# Autodesk Inventor assembly: Shooter Curve Assembly
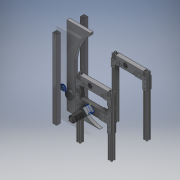
[picture p0: Inventor's stored thumbnail of the model, 180x180]
Saved by Autodesk Inventor 2018 (Build 220112000, 112)
## iProperties
Created: 2020-02-01
Part Number: Shooter Curve Assembly
Document SubType Name: Assembly
Designer: Weeb No1
Author: Weeb No1
## Documents named in this file (12)
- C:\Users\T3500STATIC\Documents\GitHub\2020CAD\Gabriel Inventor Files (Shooter, Drivebase)\Shooter Curve Assembly\Main Assembly File\Shooter Curve Assembly.iam
- C:\Users\T3500STATIC\Documents\GitHub\2020CAD\Gabriel Inventor Files (Shooter, Drivebase)\Shooter Curve Assembly\Part Files\Shooter Main Curve.ipt
- C:\Users\T3500STATIC\Documents\GitHub\2020CAD\Gabriel Inventor Files (Shooter, Drivebase)\Shooter Curve Assembly\Part Files\8020 1010 x 15.ipt
- C:\Users\T3500STATIC\Documents\GitHub\2020CAD\Gabriel Inventor Files (Shooter, Drivebase)\Shooter Curve Assembly\Part Files\1x2 5 in Beam Flywheel Mount.ipt
- C:\Users\T3500STATIC\Documents\GitHub\2020CAD\Over bumper intake\Parts\VersaPlanetary_v2_Single_Stage_10_1_with_775_Series.iam
- C:\Users\T3500STATIC\Documents\GitHub\2020CAD\Gabriel Inventor Files (Shooter, Drivebase)\Shooter Curve Assembly\Part Files\1x2 7 in Beam Motor Mount.ipt
- C:\Users\T3500STATIC\Documents\GitHub\2020CAD\Gabriel Inventor Files (Shooter, Drivebase)\Gussets\L-Gusset 3 Hole 0.25in Hole.ipt
- C:\Users\T3500STATIC\Documents\GitHub\2020CAD\Gabriel Inventor Files (Shooter, Drivebase)\Shooter Curve Assembly\Part Files\1x1 20 in Curve Support Beam.ipt
- C:\Users\T3500STATIC\Documents\GitHub\2020CAD\Gabriel Inventor Files (Shooter, Drivebase)\Gussets\L-Guesset 4 Hole 0.25in Hole.ipt
- C:\Users\T3500STATIC\Documents\GitHub\2020CAD\Gabriel Inventor Files (Shooter, Drivebase)\Gussets\L-Guesset 5 Hole 0.25in Hole.ipt
- C:\Users\T3500STATIC\Documents\GitHub\2020CAD\Gabriel Inventor Files (Shooter, Drivebase)\Shooter Curve Assembly\Part Files\_18t_Aluminum_Hub_Sprocket_25_Chain_1_2_Hex_Bore_217-3488.ipt
- C:\Users\T3500STATIC\Documents\GitHub\2020CAD\Gabriel Inventor Files (Shooter, Drivebase)\Shooter Curve Assembly\Part Files\2_OD_Straight_Flex_Wheel_217-6354.ipt
## Components (32 placed, 11 different names)
1. Shooter Main Curve:1 — Flush:1, Mate:1, Mate:2, Flush:2, Flush:3, Flush:18, Flush:20, Mate:68, Flush:36, Flush:37, Flush:40, Flush:41, Mate:133
2. 8020 1010 x 15:1 — Flush:1, Mate:1, Flush:5, Flush:6, Mate:7, Flush:11, Flush:14, Flush:18, Flush:23, Flush:24, Mate:51, Mate:56, Mate:60, Mate:82, Mate:85, Mate:97, Mate:100
3. 8020 1010 x 15:2 — Flush:4, Mate:3, Flush:7, Mate:9, Flush:15, Flush:19, Flush:22, Flush:25, Mate:127, Mate:130
4. Shooter Main Curve:2 — Mate:2, Flush:2, Flush:3, Flush:4, Mate:3, Flush:19, Flush:21, Mate:67, Flush:35, Flush:38, Flush:39, Mate:132
5. 8020 1010 x 15:3 — Flush:5, Flush:6, Flush:10, Flush:12, Flush:13, Flush:20, Mate:11, Flush:23, Mate:50, Flush:34, Mate:63, Mate:65, Mate:89, Mate:93, Mate:103, Mate:123
6. 8020 1010 x 15:4 — Flush:7, Flush:10, Flush:17, Flush:21, Mate:10, Flush:22, Mate:107, Mate:111
7. 1x2 5 in Beam Flywheel Mount:1 — Mate:9, Flush:15, Flush:17, Mate:10, Flush:25, Mate:106, Mate:108, Mate:109, Mate:110, Mate:112, Mate:113, Mate:126, Mate:128, Mate:129, Mate:131
8. 1x2 5 in Beam Flywheel Mount:2 — Mate:7, Flush:11, Flush:12, Flush:13, Flush:14, Mate:11, Flush:24, Mate:55, Mate:57, Mate:58, Mate:59, Mate:61, Mate:62, Mate:64, Mate:66
9. VersaPlanetary_v2_Single_Stage_10_1_with_775_Series:1 [sub-assembly] — Mate:52, Mate:53, Mate:54
10. 1x2 7 in Beam Motor Mount:1 — Mate:50, Mate:51, Flush:34, Mate:52, Mate:53, Mate:54, Mate:81, Mate:83, Mate:86, Mate:87, Mate:88, Mate:90, Mate:91, Mate:92, Mate:94, Mate:95, Mate:96, Mate:98, Mate:99, Mate:101, Mate:102, Mate:104, Mate:105, Mate:122, Mate:124, Mate:125
11. L-Gusset 3 Hole 0.25in Hole:1 — Mate:61, Mate:62, Mate:63
12. L-Gusset 3 Hole 0.25in Hole:2 — Mate:55, Mate:56, Mate:57
13. L-Gusset 3 Hole 0.25in Hole:3 — Mate:58, Mate:59, Mate:60
14. L-Gusset 3 Hole 0.25in Hole:4 — Mate:64, Mate:65, Mate:66
15. 1x1 20 in Curve Support Beam:1 — Mate:68, Flush:36, Flush:37
16. 1x1 20 in Curve Support Beam:2 — Mate:67, Flush:35, Flush:38
17. L-Guesset 4 Hole 0.25in Hole:3 — Mate:88, Mate:89, Mate:90, Mate:91
18. L-Guesset 4 Hole 0.25in Hole:5 — Mate:81, Mate:82, Mate:83
19. L-Guesset 4 Hole 0.25in Hole:6 — Mate:85, Mate:86, Mate:87
20. L-Guesset 4 Hole 0.25in Hole:9 — Mate:92, Mate:93, Mate:94, Mate:95
21. L-Gusset 3 Hole 0.25in Hole:9 — Mate:96, Mate:97, Mate:98
22. L-Gusset 3 Hole 0.25in Hole:10 — Mate:99, Mate:100, Mate:101
23. L-Guesset 5 Hole 0.25in Hole:1 — Mate:102, Mate:103, Mate:104, Mate:105
24. L-Guesset 5 Hole 0.25in Hole:2 — Mate:110, Mate:111, Mate:112, Mate:113
25. L-Guesset 5 Hole 0.25in Hole:3 — Mate:106, Mate:107, Mate:108, Mate:109
26. L-Guesset 5 Hole 0.25in Hole:6 — Mate:122, Mate:123, Mate:124, Mate:125
27. L-Gusset 3 Hole 0.25in Hole:11 — Mate:126, Mate:127, Mate:128
28. L-Gusset 3 Hole 0.25in Hole:12 — Mate:129, Mate:130, Mate:131
29. _18t_Aluminum_Hub_Sprocket_25_Chain_1_2_Hex_Bore_217-3488:1
30. Shooter Main Curve:4 — Flush:39, Flush:40, Flush:41, Mate:132, Mate:133
31. 2_OD_Straight_Flex_Wheel_217-6354:1
32. 2_OD_Straight_Flex_Wheel_217-6354:2
## Relationships (100: Mate 70, Flush 30)
- Flush:1 (177.8 mm): Shooter Main Curve:1 ↔ 8020 1010 x 15:1
- Mate:1 (25.4 mm): Shooter Main Curve:1 ↔ 8020 1010 x 15:1
- Mate:2 (114.3 mm): Shooter Main Curve:1 ↔ Shooter Main Curve:2
- Flush:2: Shooter Main Curve:1 ↔ Shooter Main Curve:2
- Flush:3: Shooter Main Curve:1 ↔ Shooter Main Curve:2
- Flush:4 (177.8 mm): 8020 1010 x 15:2 ↔ Shooter Main Curve:2
- Mate:3 (25.4 mm): 8020 1010 x 15:2 ↔ Shooter Main Curve:2
- Flush:5: 8020 1010 x 15:1 ↔ 8020 1010 x 15:3
- Flush:6: 8020 1010 x 15:1 ↔ 8020 1010 x 15:3
- Flush:7: 8020 1010 x 15:2 ↔ 8020 1010 x 15:4
- Flush:10: 8020 1010 x 15:3 ↔ 8020 1010 x 15:4
- Mate:7: 8020 1010 x 15:1 ↔ 1x2 5 in Beam Flywheel Mount:2
- Flush:11: 8020 1010 x 15:1 ↔ 1x2 5 in Beam Flywheel Mount:2
- Flush:12: 8020 1010 x 15:3 ↔ 1x2 5 in Beam Flywheel Mount:2
- Flush:13: 8020 1010 x 15:3 ↔ 1x2 5 in Beam Flywheel Mount:2
- Flush:14: 8020 1010 x 15:1 ↔ 1x2 5 in Beam Flywheel Mount:2
- Mate:9: 8020 1010 x 15:2 ↔ 1x2 5 in Beam Flywheel Mount:1
- Flush:15: 8020 1010 x 15:2 ↔ 1x2 5 in Beam Flywheel Mount:1
- Flush:17: 8020 1010 x 15:4 ↔ 1x2 5 in Beam Flywheel Mount:1
- Flush:18 (-25.4 mm): Shooter Main Curve:1 ↔ 8020 1010 x 15:1
- Flush:19 (-25.4 mm): 8020 1010 x 15:2 ↔ Shooter Main Curve:2
- Flush:20 (-25.4 mm): Shooter Main Curve:1 ↔ 8020 1010 x 15:3
- Flush:21 (-25.4 mm): Shooter Main Curve:2 ↔ 8020 1010 x 15:4
- Mate:10: 8020 1010 x 15:4 ↔ 1x2 5 in Beam Flywheel Mount:1
- Mate:11: 8020 1010 x 15:3 ↔ 1x2 5 in Beam Flywheel Mount:2
- Flush:22: 8020 1010 x 15:2 ↔ 8020 1010 x 15:4
- Flush:23: 8020 1010 x 15:1 ↔ 8020 1010 x 15:3
- Flush:24: 8020 1010 x 15:1 ↔ 1x2 5 in Beam Flywheel Mount:2
- Flush:25: 8020 1010 x 15:2 ↔ 1x2 5 in Beam Flywheel Mount:1
- Mate:50: 8020 1010 x 15:3 ↔ 1x2 7 in Beam Motor Mount:1
- Mate:51: 8020 1010 x 15:1 ↔ 1x2 7 in Beam Motor Mount:1
- Flush:34: 8020 1010 x 15:3 ↔ 1x2 7 in Beam Motor Mount:1
- Mate:52: VersaPlanetary_v2_Single_Stage_10_1_with_775_Series:1 ↔ 1x2 7 in Beam Motor Mount:1
- Mate:53: VersaPlanetary_v2_Single_Stage_10_1_with_775_Series:1 ↔ 1x2 7 in Beam Motor Mount:1
- Mate:54: VersaPlanetary_v2_Single_Stage_10_1_with_775_Series:1 ↔ 1x2 7 in Beam Motor Mount:1
- Mate:55: 1x2 5 in Beam Flywheel Mount:2 ↔ L-Gusset 3 Hole 0.25in Hole:2
- Mate:56: 8020 1010 x 15:1 ↔ L-Gusset 3 Hole 0.25in Hole:2
- Mate:57: 1x2 5 in Beam Flywheel Mount:2 ↔ L-Gusset 3 Hole 0.25in Hole:2
- Mate:58: 1x2 5 in Beam Flywheel Mount:2 ↔ L-Gusset 3 Hole 0.25in Hole:3
- Mate:59: 1x2 5 in Beam Flywheel Mount:2 ↔ L-Gusset 3 Hole 0.25in Hole:3
- Mate:60: 8020 1010 x 15:1 ↔ L-Gusset 3 Hole 0.25in Hole:3
- Mate:61: 1x2 5 in Beam Flywheel Mount:2 ↔ L-Gusset 3 Hole 0.25in Hole:1
- Mate:62: 1x2 5 in Beam Flywheel Mount:2 ↔ L-Gusset 3 Hole 0.25in Hole:1
- Mate:63: 8020 1010 x 15:3 ↔ L-Gusset 3 Hole 0.25in Hole:1
- Mate:64: 1x2 5 in Beam Flywheel Mount:2 ↔ L-Gusset 3 Hole 0.25in Hole:4
- Mate:65: 8020 1010 x 15:3 ↔ L-Gusset 3 Hole 0.25in Hole:4
- Mate:66: 1x2 5 in Beam Flywheel Mount:2 ↔ L-Gusset 3 Hole 0.25in Hole:4
- Mate:67: Shooter Main Curve:2 ↔ 1x1 20 in Curve Support Beam:2
- Flush:35 (-25.4 mm): Shooter Main Curve:2 ↔ 1x1 20 in Curve Support Beam:2
- Mate:68: Shooter Main Curve:1 ↔ 1x1 20 in Curve Support Beam:1
- Flush:36 (-25.4 mm): Shooter Main Curve:1 ↔ 1x1 20 in Curve Support Beam:1
- Flush:37: Shooter Main Curve:1 ↔ 1x1 20 in Curve Support Beam:1
- Flush:38: Shooter Main Curve:2 ↔ 1x1 20 in Curve Support Beam:2
- Mate:81: 1x2 7 in Beam Motor Mount:1 ↔ L-Guesset 4 Hole 0.25in Hole:5
- Mate:82: 8020 1010 x 15:1 ↔ L-Guesset 4 Hole 0.25in Hole:5
- Mate:83: 1x2 7 in Beam Motor Mount:1 ↔ L-Guesset 4 Hole 0.25in Hole:5
- Mate:85: 8020 1010 x 15:1 ↔ L-Guesset 4 Hole 0.25in Hole:6
- Mate:86: 1x2 7 in Beam Motor Mount:1 ↔ L-Guesset 4 Hole 0.25in Hole:6
- Mate:87: 1x2 7 in Beam Motor Mount:1 ↔ L-Guesset 4 Hole 0.25in Hole:6
- Mate:88: 1x2 7 in Beam Motor Mount:1 ↔ L-Guesset 4 Hole 0.25in Hole:3
- Mate:89: 8020 1010 x 15:3 ↔ L-Guesset 4 Hole 0.25in Hole:3
- Mate:90: 1x2 7 in Beam Motor Mount:1 ↔ L-Guesset 4 Hole 0.25in Hole:3
- Mate:91: 1x2 7 in Beam Motor Mount:1 ↔ L-Guesset 4 Hole 0.25in Hole:3
- Mate:92: 1x2 7 in Beam Motor Mount:1 ↔ L-Guesset 4 Hole 0.25in Hole:9
- Mate:93: 8020 1010 x 15:3 ↔ L-Guesset 4 Hole 0.25in Hole:9
- Mate:94: 1x2 7 in Beam Motor Mount:1 ↔ L-Guesset 4 Hole 0.25in Hole:9
- Mate:95: 1x2 7 in Beam Motor Mount:1 ↔ L-Guesset 4 Hole 0.25in Hole:9
- Mate:96: 1x2 7 in Beam Motor Mount:1 ↔ L-Gusset 3 Hole 0.25in Hole:9
- Mate:97: 8020 1010 x 15:1 ↔ L-Gusset 3 Hole 0.25in Hole:9
- Mate:98: 1x2 7 in Beam Motor Mount:1 ↔ L-Gusset 3 Hole 0.25in Hole:9
- Mate:99: 1x2 7 in Beam Motor Mount:1 ↔ L-Gusset 3 Hole 0.25in Hole:10
- Mate:100: 8020 1010 x 15:1 ↔ L-Gusset 3 Hole 0.25in Hole:10
- Mate:101: 1x2 7 in Beam Motor Mount:1 ↔ L-Gusset 3 Hole 0.25in Hole:10
- Mate:102: 1x2 7 in Beam Motor Mount:1 ↔ L-Guesset 5 Hole 0.25in Hole:1
- Mate:103: 8020 1010 x 15:3 ↔ L-Guesset 5 Hole 0.25in Hole:1
- Mate:104: 1x2 7 in Beam Motor Mount:1 ↔ L-Guesset 5 Hole 0.25in Hole:1
- Mate:105: 1x2 7 in Beam Motor Mount:1 ↔ L-Guesset 5 Hole 0.25in Hole:1
- Mate:106: 1x2 5 in Beam Flywheel Mount:1 ↔ L-Guesset 5 Hole 0.25in Hole:3
- Mate:107: 8020 1010 x 15:4 ↔ L-Guesset 5 Hole 0.25in Hole:3
- Mate:108: 1x2 5 in Beam Flywheel Mount:1 ↔ L-Guesset 5 Hole 0.25in Hole:3
- Mate:109: 1x2 5 in Beam Flywheel Mount:1 ↔ L-Guesset 5 Hole 0.25in Hole:3
- Mate:110: 1x2 5 in Beam Flywheel Mount:1 ↔ L-Guesset 5 Hole 0.25in Hole:2
- Mate:111: 8020 1010 x 15:4 ↔ L-Guesset 5 Hole 0.25in Hole:2
- Mate:112: 1x2 5 in Beam Flywheel Mount:1 ↔ L-Guesset 5 Hole 0.25in Hole:2
- Mate:113: 1x2 5 in Beam Flywheel Mount:1 ↔ L-Guesset 5 Hole 0.25in Hole:2
- Mate:122: 1x2 7 in Beam Motor Mount:1 ↔ L-Guesset 5 Hole 0.25in Hole:6
- Mate:123: 8020 1010 x 15:3 ↔ L-Guesset 5 Hole 0.25in Hole:6
- Mate:124: 1x2 7 in Beam Motor Mount:1 ↔ L-Guesset 5 Hole 0.25in Hole:6
- Mate:125: 1x2 7 in Beam Motor Mount:1 ↔ L-Guesset 5 Hole 0.25in Hole:6
- Mate:126: 1x2 5 in Beam Flywheel Mount:1 ↔ L-Gusset 3 Hole 0.25in Hole:11
- Mate:127: 8020 1010 x 15:2 ↔ L-Gusset 3 Hole 0.25in Hole:11
- Mate:128: 1x2 5 in Beam Flywheel Mount:1 ↔ L-Gusset 3 Hole 0.25in Hole:11
- Mate:129: 1x2 5 in Beam Flywheel Mount:1 ↔ L-Gusset 3 Hole 0.25in Hole:12
- Mate:130: 8020 1010 x 15:2 ↔ L-Gusset 3 Hole 0.25in Hole:12
- Mate:131: 1x2 5 in Beam Flywheel Mount:1 ↔ L-Gusset 3 Hole 0.25in Hole:12
- Flush:39: Shooter Main Curve:2 ↔ Shooter Main Curve:4
- Flush:40: Shooter Main Curve:1 ↔ Shooter Main Curve:4
- Flush:41: Shooter Main Curve:1 ↔ Shooter Main Curve:4
- Mate:132 (47.625 mm): Shooter Main Curve:2 ↔ Shooter Main Curve:4
- Mate:133 (47.625 mm): Shooter Main Curve:1 ↔ Shooter Main Curve:4
